# Autodesk Inventor assembly: modul
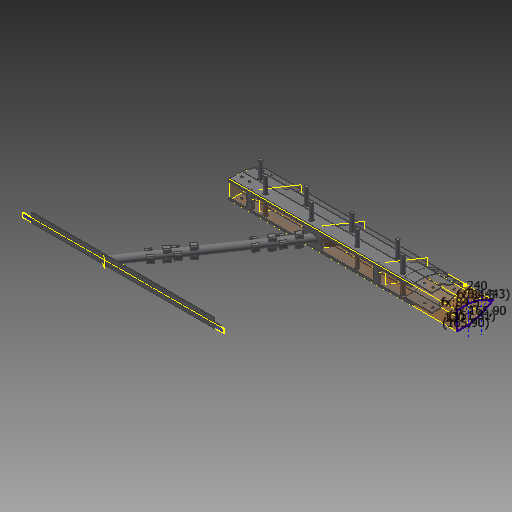
[picture p0: Inventor's stored thumbnail of the model, 512x512]
Saved by Autodesk Inventor 2018 (Build 220112000, 112)
## iProperties
Created: 2019-09-23
Part Number: modul
Document SubType Name: Assembly
Designer: loppen
Mass: 37010.5 g
Surface Area: 22000.8 cm^2
Volume: 4857.58 cm^3
Density: 7.61912 g/cm^3
Author: loppen
## Documents named in this file (19)
- Z:\trappe\modul.iam
- Z:\trappe\model.ipt
- Z:\trappe\vange.ipt
- Z:\trappe\baluster\stilladssøjle.iam
- Z:\trappe\baluster-fod.ipt
- Z:\trappe\håndfang\håndfang.iam
- Z:\trappe\trappestift skrå.ipt
- Z:\trappe\trappestift.ipt
- Z:\trappe\laske.ipt
- Z:\trappe\laske spejlet.ipt
- Z:\trappe\skot.ipt
- Z:\trappe\skot opad.ipt
- Z:\trappe\modul\AIP\FEA\d09v3y4ww.fins
- Z:\trappe\modul\AIP\FEA\d09v3y4ww.fsat
- Z:\trappe\modul\AIP\FEA\d09v3y4ww.ftes
- Z:\trappe\modul\AIP\FEA\d09v3y4ww.fwiz
- Z:\trappe\modul\AIP\FEA\d09v3y50g.fmsh
- Z:\trappe\modul\AIP\FEA\d09v3y50h.fres
- Z:\trappe\trappe.xlsx
## Components (19 placed, 11 different names)
1. model:1 — Flush:1, Flush:2, Flush:3, Flush:4, Flush:5, Flush:6, Flush:7, Flush:8
2. vange:1 — Flush:1, Flush:2, Flush:3, Flush:4, Flush:5, Flush:6, Flush:7, Flush:8, Mate:1, Flush:9, Mate:3, Flush:11, Mate:7, Mate:8, Mate:9, Mate:10, Mate:11, Mate:12, Mate:13, Mate:14, Angle:1, Angle:2, Angle:3, Angle:4, Angle:5, Angle:6, Angle:7, Angle:8, Flush:12, Flush:13, Flush:14, Flush:15, Mate:15, Mate:16, Mate:17, Mate:18, Mate:21, Mate:22, Mate:23, Mate:24, Mate:25, Mate:26, Mate:27, Mate:28, Mate:29, Mate:30, Mate:31, Mate:32, Flush:18, Flush:19, Flush:20, Flush:21
3. stilladssøjle:1 [sub-assembly] — Mate:1, Flush:9, Flush:10, Mate:2, Mate:4, Mate:5, Mate:6
4. baluster-fod:1 — Flush:10, Mate:2, Mate:3, Mate:4, Flush:16, Flush:17
5. håndfang:1 [sub-assembly] — Mate:5, Flush:11, Mate:6
6. trappestift skrå:1 — Mate:7, Angle:1, Mate:15
7. trappestift:1 — Mate:8, Angle:2, Flush:12
8. trappestift skrå:3 — Mate:9, Angle:3, Mate:16
9. trappestift:2 — Mate:10, Angle:4, Flush:13
10. trappestift skrå:5 — Mate:11, Angle:5, Mate:17
11. trappestift:3 — Mate:12, Angle:6, Flush:14
12. trappestift skrå:7 — Mate:13, Angle:7, Mate:18
13. trappestift:4 — Mate:14, Angle:8, Flush:15
14. laske:2 — Mate:21, Mate:22, Mate:23
15. laske spejlet:1 — Mate:24, Mate:25, Mate:26
16. skot:1 — Mate:27, Mate:28, Flush:16
17. skot:2 — Mate:29, Mate:30, Flush:17
18. skot opad:1 — Mate:31, Flush:19, Flush:20
19. skot opad:2 — Mate:32, Flush:18, Flush:21
## Relationships (59: Mate 30, Flush 21, Angle 8)
- Flush:1: model:1 ↔ vange:1
- Flush:2: model:1 ↔ vange:1
- Flush:3: model:1 ↔ vange:1
- Flush:4: model:1 ↔ vange:1
- Flush:5: model:1 ↔ vange:1
- Flush:6: model:1 ↔ vange:1
- Flush:7: model:1 ↔ vange:1
- Flush:8: model:1 ↔ vange:1
- Mate:1: vange:1 ↔ stilladssøjle:1
- Flush:9: vange:1 ↔ stilladssøjle:1
- Flush:10: stilladssøjle:1 ↔ baluster-fod:1
- Mate:2: stilladssøjle:1 ↔ baluster-fod:1
- Mate:3 (43.655 mm): vange:1 ↔ baluster-fod:1
- Mate:4: stilladssøjle:1 ↔ baluster-fod:1
- Mate:5: stilladssøjle:1 ↔ håndfang:1
- Flush:11: vange:1 ↔ håndfang:1
- Mate:6 (-90 mm): stilladssøjle:1 ↔ håndfang:1
- Mate:7: vange:1 ↔ trappestift skrå:1
- Mate:8: vange:1 ↔ trappestift:1
- Mate:9: vange:1 ↔ trappestift skrå:3
- Mate:10: vange:1 ↔ trappestift:2
- Mate:11: vange:1 ↔ trappestift skrå:5
- Mate:12: vange:1 ↔ trappestift:3
- Mate:13: vange:1 ↔ trappestift skrå:7
- Mate:14: vange:1 ↔ trappestift:4
- Angle:1 (0 deg): vange:1 ↔ trappestift skrå:1
- Angle:2 (0 deg): vange:1 ↔ trappestift:1
- Angle:3 (0 deg): vange:1 ↔ trappestift skrå:3
- Angle:4 (0 deg): vange:1 ↔ trappestift:2
- Angle:5 (0 deg): vange:1 ↔ trappestift skrå:5
- Angle:6 (0 deg): vange:1 ↔ trappestift:3
- Angle:7 (0 deg): vange:1 ↔ trappestift skrå:7
- Angle:8 (0 deg): vange:1 ↔ trappestift:4
- Flush:12: vange:1 ↔ trappestift:1
- Flush:13: vange:1 ↔ trappestift:2
- Flush:14: vange:1 ↔ trappestift:3
- Flush:15: vange:1 ↔ trappestift:4
- Mate:15: vange:1 ↔ trappestift skrå:1
- Mate:16: vange:1 ↔ trappestift skrå:3
- Mate:17: vange:1 ↔ trappestift skrå:5
- Mate:18: vange:1 ↔ trappestift skrå:7
- Mate:21: vange:1 ↔ laske:2
- Mate:22: vange:1 ↔ laske:2
- Mate:23 (32.5 mm): vange:1 ↔ laske:2
- Mate:24: vange:1 ↔ laske spejlet:1
- Mate:25: vange:1 ↔ laske spejlet:1
- Mate:26 (32.5 mm): vange:1 ↔ laske spejlet:1
- Mate:27: vange:1 ↔ skot:1
- Mate:28 (1.659 mm): vange:1 ↔ skot:1
- Flush:16 (345.087 mm): baluster-fod:1 ↔ skot:1
- Mate:29: vange:1 ↔ skot:2
- Mate:30 (1.659 mm): vange:1 ↔ skot:2
- Flush:17 (-345.087 mm): baluster-fod:1 ↔ skot:2
- Mate:31 (2 mm): vange:1 ↔ skot opad:1
- Mate:32 (2 mm): vange:1 ↔ skot opad:2
- Flush:18 (13.5 mm): vange:1 ↔ skot opad:2
- Flush:19 (13.5 mm): vange:1 ↔ skot opad:1
- Flush:20: vange:1 ↔ skot opad:1
- Flush:21: vange:1 ↔ skot opad:2
## Named parameters: sa_0 = 0, sa_1 = 0, sa_2 = -250000, trappestifter_dia = 25 mm, trappestifter_laengde = 228 mm, perforeringsbredde = 6 mm, perforeringshulprocent = 80 mm, perforeringshullaengde = 62.8 mm, perforeringsoffset = 8 mm, perforeringsoffset_top = 8 mm, perforeringsoffset_bund = 8 mm, laskehul_dia = 13 mm, perforeringshullaengde_top = 61 mm, perforeringshullaengde_bund = 61.6 mm, trappestifter_huldia = 25.8 mm, trappestifter_skraa_huldia = 26.6 mm, håndfang_offset_fra_top = 70 mm, haandfang_offset_fra_top = 90 mm, trappevinkel = 34.3 deg, balusterhul_udvidelse = 1 mm, pladetykkelse = 3 mm
note: some values were not read from the file. Shown as the stored number, unit unknown: "sa_0", "sa_1", "sa_2".
